# Autodesk Inventor assembly: MechSwitch_Assem_V2
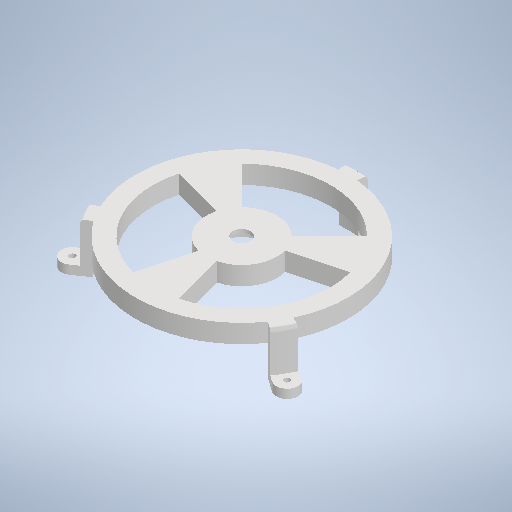
[picture p0: Inventor's stored thumbnail of the model, 512x512]
Saved by Autodesk Inventor 2025.1 (Build 291241000, 241)
## iProperties
Created: 2026-04-13
Part Number: MechSwitch_Assem_V2
Document SubType Name: Assembly
Designer: ryand
Author: ryand
## Documents named in this file (4)
- C:\Users\ryand\OneDrive\Documents\Inventor\TNG\Rotational_TENG\MechSwitch\MechSwitch_Assem_V2.iam
- C:\Users\ryand\OneDrive\Documents\Inventor\TNG\Rotational_TENG\MechSwitch\MechSwitch_DielecTopV2.ipt
- C:\Users\ryand\OneDrive\Documents\Inventor\TNG\Rotational_TENG\MechSwitch\Bearing-Insert.ipt
- C:\Users\ryand\OneDrive\Documents\Inventor\TNG\Rotational_TENG\MechSwitch\PCB_insert.ipt
## Components (3 placed, 3 different names)
1. MechSwitch_DielecTopV2:1 — Mate:3
2. Bearing-Insert:1 — Mate:3
3. PCB_insert:1
## Relationships (1: Mate 1)
- Mate:3: MechSwitch_DielecTopV2:1 ↔ Bearing-Insert:1
